# Autodesk Inventor assembly: Assembly1
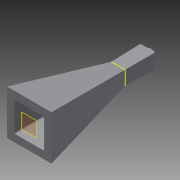
[picture p0: Inventor's stored thumbnail of the model, 180x180]
Saved by Autodesk Inventor 2018.2 (Build 222227000, 227)
## iProperties
Created: 2018-02-02
Part Number: Assembly1
Document SubType Name: Assembly
Designer: Rus
Author: Rus
## Documents named in this file (6)
- E:\Libraries\3D Objects\Air Raid\V0\Assembly1.iam
- E:\Libraries\3D Objects\Air Raid\V0\Impeller.ipt
- E:\Libraries\3D Objects\Air Raid\V0\Stator.ipt
- E:\Libraries\3D Objects\Air Raid\V0\1inch wide turbo.ipt
- E:\Libraries\3D Objects\Air Raid\V0\Stator Front.ipt
- E:\Libraries\3D Objects\Air Raid\V0\WindHelper.ipt
## Components (5 placed, 5 different names)
1. Impeller:1 — Insert:1, Angle:1, Insert:2
2. Stator:1 — Insert:1, Insert:3, Tangent:1
3. 1inch wide turbo:1 — Angle:1, Insert:2
4. Stator Front:1 — Insert:3, Tangent:1, Insert:4
5. WindHelper:1 — Insert:4
## Relationships (6: Insert 4, Angle 1, Tangent 1)
- Insert:1: Impeller:1 ↔ Stator:1
- Angle:1 (0 deg): Impeller:1 ↔ 1inch wide turbo:1
- Insert:2: Impeller:1 ↔ 1inch wide turbo:1
- Insert:3: Stator:1 ↔ Stator Front:1
- Tangent:1: Stator:1 ↔ Stator Front:1
- Insert:4: Stator Front:1 ↔ WindHelper:1
